# Autodesk Inventor assembly: RC_CAR_CHASSIS
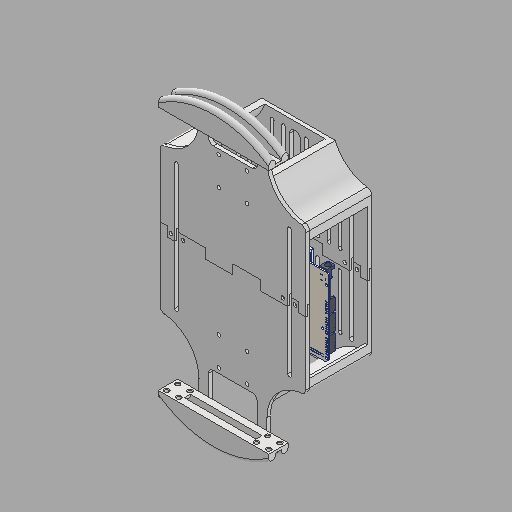
[picture p0: Inventor's stored thumbnail of the model, 512x512]
Saved by Autodesk Inventor 2025.2 (Build 292293000, 293)
## iProperties
Created: 2025-10-27
Part Number: RC_CAR_CHASSIS
Document SubType Name: Assembly
Designer: Ben
Author: Ben
## Documents named in this file (6)
- C:\Users\Ben\3D Objects\3 RC_CAR\RC_CAR_CHASSIS.iam
- C:\Users\Ben\3D Objects\3 RC_CAR\RC_CAR_BUMPER.ipt
- C:\Users\Ben\3D Objects\3 RC_CAR\RC_CAR_BASE_PLATE.ipt
- C:\Users\Ben\3D Objects\3 RC_CAR\RC_CAR_CONTROLLER_PLATE.ipt
- C:\Users\Ben\3D Objects\3 RC_CAR\RC_CAR_TOP_PLATE.ipt
- C:\Users\Ben\Downloads\arduino-mega-2560-8.snapshot.1\Arduino Mega 2560\Arduino Mega 2560\Arduino Mega 2560.ipt
## Components (8 placed, 5 different names)
1. RC_CAR_BUMPER:1 — Insert:1, Insert:2
2. RC_CAR_BUMPER:2 — Insert:5, Insert:6
3. RC_CAR_BASE_PLATE:1 — Insert:1, Insert:2, Insert:3, Insert:4, Tangent:1, Insert:10, Insert:11
4. RC_CAR_BASE_PLATE:2 — Insert:3, Insert:4, Insert:5, Insert:6, Mate:1, Tangent:2, Angle:1, Insert:7, Insert:12, Angle:2
5. RC_CAR_CONTROLLER_PLATE:1 — Tangent:1, Mate:1, Tangent:2, Angle:1, Mate:2
6. RC_CAR_TOP_PLATE:1 — Insert:7, Insert:12
7. RC_CAR_TOP_PLATE:2 — Insert:10, Insert:11
8. Arduino Mega 2560:1 — Mate:2, Angle:2
## Relationships (16: Insert 10, Tangent 2, Mate 2, Angle 2)
- Insert:1: RC_CAR_BUMPER:1 ↔ RC_CAR_BASE_PLATE:1
- Insert:2: RC_CAR_BUMPER:1 ↔ RC_CAR_BASE_PLATE:1
- Insert:3: RC_CAR_BASE_PLATE:1 ↔ RC_CAR_BASE_PLATE:2
- Insert:4: RC_CAR_BASE_PLATE:1 ↔ RC_CAR_BASE_PLATE:2
- Insert:5: RC_CAR_BUMPER:2 ↔ RC_CAR_BASE_PLATE:2
- Insert:6: RC_CAR_BUMPER:2 ↔ RC_CAR_BASE_PLATE:2
- Tangent:1: RC_CAR_BASE_PLATE:1 ↔ RC_CAR_CONTROLLER_PLATE:1
- Mate:1: RC_CAR_BASE_PLATE:2 ↔ RC_CAR_CONTROLLER_PLATE:1
- Tangent:2: RC_CAR_BASE_PLATE:2 ↔ RC_CAR_CONTROLLER_PLATE:1
- Angle:1 (0 deg): RC_CAR_BASE_PLATE:2 ↔ RC_CAR_CONTROLLER_PLATE:1
- Insert:7: RC_CAR_BASE_PLATE:2 ↔ RC_CAR_TOP_PLATE:1
- Insert:10: RC_CAR_BASE_PLATE:1 ↔ RC_CAR_TOP_PLATE:2
- Insert:11: RC_CAR_BASE_PLATE:1 ↔ RC_CAR_TOP_PLATE:2
- Insert:12: RC_CAR_BASE_PLATE:2 ↔ RC_CAR_TOP_PLATE:1
- Mate:2 (25.4 mm): RC_CAR_CONTROLLER_PLATE:1 ↔ Arduino Mega 2560:1
- Angle:2 (180 deg): RC_CAR_BASE_PLATE:2 ↔ Arduino Mega 2560:1
